# Autodesk Inventor assembly: assembly_testing lcd
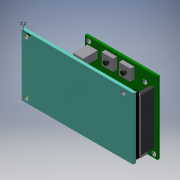
[picture p0: Inventor's stored thumbnail of the model, 180x180]
Saved by Autodesk Inventor 2017 (Build 210142000, 142)
## iProperties
Created: 2016-11-07
Part Number: assembly_testing lcd
Document SubType Name: Assembly
Designer: radrajith
Author: radrajith
## Documents named in this file (3)
- C:\Users\radra\Box Sync\Senior Fall 2016\ESE 323\autocad\assembly_testing lcd.iam
- C:\Users\radra\Box Sync\Senior Fall 2016\ESE 323\autocad\lab 04.ipt
- C:\Users\radra\Box Sync\Senior Fall 2016\ESE 323\autocad\lcd display.ipt
## Components (2 placed, 2 different names)
1. lab 04:1 — Mate:1, Mate:2
2. lcd display:1 — Mate:1, Mate:2
## Relationships (2: Mate 2)
- Mate:1: lab 04:1 ↔ lcd display:1
- Mate:2: lab 04:1 ↔ lcd display:1
